# Autodesk Inventor assembly: top-idler
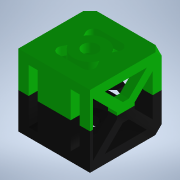
[picture p0: Inventor's stored thumbnail of the model, 180x180]
Saved by Autodesk Inventor 2020.4 (Build 244396000, 396)
## iProperties
Created: 2021-04-07
Part Number: top-idler
Document SubType Name: Assembly
Designer: AOB
Mass: 5.77904 g
Surface Area: 58.3557 cm^2
Volume: 5.45193 cm^3
Density: 1.06 g/cm^3
Author: AOB
## Documents named in this file (2)
- C:\Users\marti\Documents\Inventor\ProjectBoron\Boron Ultima\top-idler.iam
- C:\Users\marti\Documents\Inventor\ProjectBoron\Boron Ultima\top-idler V2.ipt
## Components (2 placed, 1 different names)
1. top-idler V2:1 — Flush:1, Flush:2, Rigid:1
2. top-idler V2:2 — Flush:1, Flush:2, Rigid:1
## Relationships (3: Flush 2, WeldJoint 1)
- Flush:1: top-idler V2:1 ↔ top-idler V2:2
- Flush:2: top-idler V2:1 ↔ top-idler V2:2
- Rigid:1 [WeldJoint]: top-idler V2:1 ↔ top-idler V2:2
